# Autodesk Inventor assembly: Head
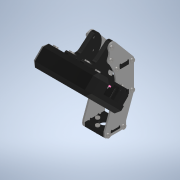
[picture p0: Inventor's stored thumbnail of the model, 180x180]
Saved by Autodesk Inventor 2020.4 (Build 244396000, 396)
## iProperties
Created: 2021-09-05
Part Number: Head
Document SubType Name: Assembly
Designer: Masato
Mass: 100.328 g
Surface Area: 575.675 cm^2
Volume: 96.16 cm^3
Density: 1.04334 g/cm^3
Author: Masato
## Documents named in this file (12)
- C:\Users\Masato\Documents\Inventor\CIT Brains_Inventor\OpenPlatform_ver3_0 - ve4_1 branch\UpperBody\Head\Head.iam
- C:\Users\Masato\Documents\Inventor\CIT Brains_Inventor\OpenPlatform_ver3_0 - ve4_1 branch\Ready_Made\KBCR-S02MU.ipt
- C:\Users\Masato\Documents\Inventor\CIT Brains_Inventor\OpenPlatform_ver3_0 - ve4_1 branch\UpperBody\Head\Camera_side_frame.ipt
- C:\Users\Masato\Documents\Inventor\CIT Brains_Inventor\OpenPlatform_ver3_0 - ve4_1 branch\UpperBody\Head\Camera_root_frame.ipt
- C:\Users\Masato\Documents\Inventor\CIT Brains_Inventor\OpenPlatform_ver3_0 - ve4_1 branch\UpperBody\Head\Camera_cover.ipt
- C:\Users\Masato\Documents\Inventor\CIT Brains_Inventor\OpenPlatform_ver3_0 - ve4_1 branch\UpperBody\Head\Head_horn_frame.ipt
- C:\Users\Masato\Documents\Inventor\CIT Brains_Inventor\OpenPlatform_ver3_0 - ve4_1 branch\UpperBody\Head\Head_diagonal.ipt
- C:\Users\Masato\Documents\Inventor\CIT Brains_Inventor\OpenPlatform_ver3_0 - ve4_1 branch\UpperBody\Head\Head_side_frame.ipt
- C:\Users\Masato\Documents\Inventor\CIT Brains_Inventor\OpenPlatform_ver3_0 - ve4_1 branch\Ready_Made\Screw\M3-6.ipt
- C:\Users\Masato\Documents\Inventor\CIT Brains_Inventor\OpenPlatform_ver3_0 - ve4_1 branch\Ready_Made\Screw\M2-6.ipt
- C:\Users\Masato\Documents\Inventor\CIT Brains_Inventor\OpenPlatform_ver3_0 - ve4_1 branch\Ready_Made\UD-43040.ipt
- C:\Users\Masato\Documents\Inventor\CIT Brains_Inventor\OpenPlatform_ver3_0 - ve4_1 branch\Ready_Made\Screw\M2_6-8.ipt
## Components (46 placed, 11 different names)
1. KBCR-S02MU:1 — 挿入:23, 挿入:24, 挿入:25, 挿入:26, 挿入:58, 挿入:59, 挿入:60, 挿入:61
2. Camera_side_frame:1 — 挿入:3, 挿入:7, 挿入:33, 挿入:50, 挿入:53
3. Camera_side_frame:2 — 挿入:5, 挿入:6, 挿入:9, 挿入:10, 挿入:51, 挿入:52
4. Camera_root_frame:1 — 挿入:3, 挿入:5, 挿入:6, 挿入:33, 挿入:23, 挿入:24, 挿入:25, 挿入:26, 挿入:54, 挿入:55, 挿入:56, 挿入:57, 挿入:71, 挿入:72
5. Camera_cover:1 — 挿入:62, 挿入:63, 挿入:64, 挿入:65
6. Head_horn_frame:1 — 挿入:29, 挿入:30, 挿入:31, 挿入:32, フラッシュ:1, フラッシュ:2, メイト:1, 挿入:67, 挿入:68, 挿入:69, 挿入:70
7. Head_diagonal:1 — 挿入:11, 挿入:12, 挿入:15, 挿入:16
8. Head_diagonal:2 — 挿入:13, 挿入:14, 挿入:17, 挿入:18
9. Head_side_frame:1 — 挿入:7, 挿入:11, 挿入:12, 挿入:13, 挿入:14, 挿入:29, 挿入:30, 挿入:34, 挿入:35, 挿入:36, 挿入:37, 挿入:38, 挿入:39, 挿入:40, 挿入:41
10. Head_side_frame:2 — 挿入:9, 挿入:10, 挿入:15, 挿入:16, 挿入:17, 挿入:18, 挿入:31, 挿入:32, 挿入:42, 挿入:43, 挿入:44, 挿入:45, 挿入:46, 挿入:47, 挿入:48, 挿入:49
11. M3-6:1 — 挿入:34
12. M3-6:2 — 挿入:35
13. M3-6:3 — 挿入:36
14. M3-6:4 — 挿入:37
15. M3-6:5 — 挿入:38
16. M3-6:6 — 挿入:39
17. M3-6:7 — 挿入:40
18. M3-6:8 — 挿入:41
19. M3-6:9 — 挿入:42
20. M3-6:10 — 挿入:43
21. M3-6:11 — 挿入:44
22. M3-6:12 — 挿入:45
23. M3-6:13 — 挿入:46
24. M3-6:14 — 挿入:47
25. M3-6:15 — 挿入:48
26. M3-6:16 — 挿入:49
27. M3-6:17 — 挿入:50
28. M3-6:18 — 挿入:51
29. M3-6:19 — 挿入:52
30. M3-6:20 — 挿入:53
31. M3-6:21 — 挿入:54
32. M3-6:22 — 挿入:55
33. M3-6:23 — 挿入:56
34. M3-6:24 — 挿入:57
35. M2-6:1 — 挿入:58
36. M2-6:2 — 挿入:59
37. M2-6:3 — 挿入:61
38. M2-6:4 — 挿入:60
39. UD-43040:1 — 挿入:62
40. UD-43040:2 — 挿入:63, 挿入:72
41. UD-43040:3 — 挿入:64, 挿入:71
42. UD-43040:4 — 挿入:65
43. M2_6-8:1 — 挿入:67
44. M2_6-8:2 — 挿入:68
45. M2_6-8:3 — 挿入:69
46. M2_6-8:4 — 挿入:70
## Relationships (64: Insert 61, Flush 2, Mate 1)
- 挿入:3 [Insert]: Camera_side_frame:1 ↔ Camera_root_frame:1
- 挿入:5 [Insert]: Camera_side_frame:2 ↔ Camera_root_frame:1
- 挿入:6 [Insert]: Camera_side_frame:2 ↔ Camera_root_frame:1
- 挿入:33 [Insert]: Camera_side_frame:1 ↔ Camera_root_frame:1
- 挿入:7 [Insert]: Camera_side_frame:1 ↔ Head_side_frame:1
- 挿入:9 [Insert]: Camera_side_frame:2 ↔ Head_side_frame:2
- 挿入:10 [Insert]: Camera_side_frame:2 ↔ Head_side_frame:2
- 挿入:11 [Insert]: Head_diagonal:1 ↔ Head_side_frame:1
- 挿入:12 [Insert]: Head_diagonal:1 ↔ Head_side_frame:1
- 挿入:13 [Insert]: Head_diagonal:2 ↔ Head_side_frame:1
- 挿入:14 [Insert]: Head_diagonal:2 ↔ Head_side_frame:1
- 挿入:15 [Insert]: Head_diagonal:1 ↔ Head_side_frame:2
- 挿入:16 [Insert]: Head_diagonal:1 ↔ Head_side_frame:2
- 挿入:17 [Insert]: Head_diagonal:2 ↔ Head_side_frame:2
- 挿入:18 [Insert]: Head_diagonal:2 ↔ Head_side_frame:2
- 挿入:23 [Insert]: KBCR-S02MU:1 ↔ Camera_root_frame:1
- 挿入:24 [Insert]: KBCR-S02MU:1 ↔ Camera_root_frame:1
- 挿入:25 [Insert]: KBCR-S02MU:1 ↔ Camera_root_frame:1
- 挿入:26 [Insert]: KBCR-S02MU:1 ↔ Camera_root_frame:1
- 挿入:29 [Insert]: Head_horn_frame:1 ↔ Head_side_frame:1
- 挿入:30 [Insert]: Head_horn_frame:1 ↔ Head_side_frame:1
- 挿入:31 [Insert]: Head_horn_frame:1 ↔ Head_side_frame:2
- 挿入:32 [Insert]: Head_horn_frame:1 ↔ Head_side_frame:2
- 挿入:34 [Insert]: Head_side_frame:1 ↔ M3-6:1
- 挿入:35 [Insert]: Head_side_frame:1 ↔ M3-6:2
- 挿入:36 [Insert]: Head_side_frame:1 ↔ M3-6:3
- 挿入:37 [Insert]: Head_side_frame:1 ↔ M3-6:4
- 挿入:38 [Insert]: Head_side_frame:1 ↔ M3-6:5
- 挿入:39 [Insert]: Head_side_frame:1 ↔ M3-6:6
- 挿入:40 [Insert]: Head_side_frame:1 ↔ M3-6:7
- 挿入:41 [Insert]: Head_side_frame:1 ↔ M3-6:8
- 挿入:42 [Insert]: Head_side_frame:2 ↔ M3-6:9
- 挿入:43 [Insert]: Head_side_frame:2 ↔ M3-6:10
- 挿入:44 [Insert]: Head_side_frame:2 ↔ M3-6:11
- 挿入:45 [Insert]: Head_side_frame:2 ↔ M3-6:12
- 挿入:46 [Insert]: Head_side_frame:2 ↔ M3-6:13
- 挿入:47 [Insert]: Head_side_frame:2 ↔ M3-6:14
- 挿入:48 [Insert]: Head_side_frame:2 ↔ M3-6:15
- 挿入:49 [Insert]: Head_side_frame:2 ↔ M3-6:16
- 挿入:50 [Insert]: Camera_side_frame:1 ↔ M3-6:17
- 挿入:51 [Insert]: Camera_side_frame:2 ↔ M3-6:18
- 挿入:52 [Insert]: Camera_side_frame:2 ↔ M3-6:19
- 挿入:53 [Insert]: Camera_side_frame:1 ↔ M3-6:20
- 挿入:54 [Insert]: Camera_root_frame:1 ↔ M3-6:21
- 挿入:55 [Insert]: Camera_root_frame:1 ↔ M3-6:22
- 挿入:56 [Insert]: Camera_root_frame:1 ↔ M3-6:23
- 挿入:57 [Insert]: Camera_root_frame:1 ↔ M3-6:24
- 挿入:58 [Insert]: KBCR-S02MU:1 ↔ M2-6:1
- 挿入:59 [Insert]: KBCR-S02MU:1 ↔ M2-6:2
- 挿入:60 [Insert]: KBCR-S02MU:1 ↔ M2-6:4
- 挿入:61 [Insert]: KBCR-S02MU:1 ↔ M2-6:3
- 挿入:62 [Insert]: Camera_cover:1 ↔ UD-43040:1
- 挿入:63 [Insert]: Camera_cover:1 ↔ UD-43040:2
- 挿入:64 [Insert]: Camera_cover:1 ↔ UD-43040:3
- 挿入:65 [Insert]: Camera_cover:1 ↔ UD-43040:4
- フラッシュ:1 [Flush]: Head_horn_frame:1
- フラッシュ:2 [Flush]: Head_horn_frame:1
- メイト:1 [Mate]: Head_horn_frame:1
- 挿入:67 [Insert]: Head_horn_frame:1 ↔ M2_6-8:1
- 挿入:68 [Insert]: Head_horn_frame:1 ↔ M2_6-8:2
- 挿入:69 [Insert]: Head_horn_frame:1 ↔ M2_6-8:3
- 挿入:70 [Insert]: Head_horn_frame:1 ↔ M2_6-8:4
- 挿入:71 [Insert]: Camera_root_frame:1 ↔ UD-43040:3
- 挿入:72 [Insert]: Camera_root_frame:1 ↔ UD-43040:2
